# Autodesk Inventor assembly: pulley 48 tooth + hub
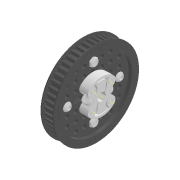
[picture p0: Inventor's stored thumbnail of the model, 180x180]
Saved by Autodesk Inventor 2020 (Build 240168000, 168)
## iProperties
Created: 2020-02-22
Part Number: pulley 48 tooth + hub
Document SubType Name: Assembly
Designer: ball
Author: ball
## Documents named in this file (4)
- C:\FTC\FTC8863CAD\2019 Robot\Mecanum Drive Train Metal\pulley 48 tooth + hub.iam
- C:\FTC\FTC8863CAD\GoBilda\3415 Parts\3415-0014-0048 Assembly.ipt
- C:\FTC\FTC8863CAD\GoBilda\1309 Parts\1309-0016-4008 assembly.ipt
- C:\FTC\FTC8863CAD\StepLibraries\Screws\M4 x 14 BUTTON HEAD HEX DRIVE SCREW.ipt
## Components (6 placed, 3 different names)
1. 3415-0014-0048 Assembly:1 — Mate:1, Mate:2, Flush:1, Mate:9, Mate:11, Mate:13, Mate:15
2. 1309-0016-4008 assembly:1 — Mate:1, Mate:2, Flush:1, Mate:10, Mate:12, Mate:14, Mate:16
3. M4 x 14 BUTTON HEAD HEX DRIVE SCREW:1 — Mate:9, Mate:10
4. M4 x 14 BUTTON HEAD HEX DRIVE SCREW:2 — Mate:11, Mate:12
5. M4 x 14 BUTTON HEAD HEX DRIVE SCREW:3 — Mate:15, Mate:16
6. M4 x 14 BUTTON HEAD HEX DRIVE SCREW:4 — Mate:13, Mate:14
## Relationships (11: Mate 10, Flush 1)
- Mate:1: 3415-0014-0048 Assembly:1 ↔ 1309-0016-4008 assembly:1
- Mate:2: 3415-0014-0048 Assembly:1 ↔ 1309-0016-4008 assembly:1
- Flush:1: 3415-0014-0048 Assembly:1 ↔ 1309-0016-4008 assembly:1
- Mate:9: 3415-0014-0048 Assembly:1 ↔ M4 x 14 BUTTON HEAD HEX DRIVE SCREW:1
- Mate:10: 1309-0016-4008 assembly:1 ↔ M4 x 14 BUTTON HEAD HEX DRIVE SCREW:1
- Mate:11: 3415-0014-0048 Assembly:1 ↔ M4 x 14 BUTTON HEAD HEX DRIVE SCREW:2
- Mate:12: 1309-0016-4008 assembly:1 ↔ M4 x 14 BUTTON HEAD HEX DRIVE SCREW:2
- Mate:13: 3415-0014-0048 Assembly:1 ↔ M4 x 14 BUTTON HEAD HEX DRIVE SCREW:4
- Mate:14: 1309-0016-4008 assembly:1 ↔ M4 x 14 BUTTON HEAD HEX DRIVE SCREW:4
- Mate:15: 3415-0014-0048 Assembly:1 ↔ M4 x 14 BUTTON HEAD HEX DRIVE SCREW:3
- Mate:16: 1309-0016-4008 assembly:1 ↔ M4 x 14 BUTTON HEAD HEX DRIVE SCREW:3
